# Autodesk Inventor assembly: 1.5 in Bottom Block WCP-0419
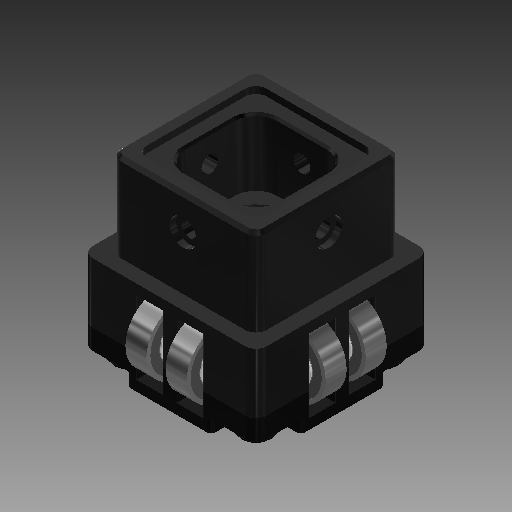
[picture p0: Inventor's stored thumbnail of the model, 512x512]
Saved by Autodesk Inventor 2023 (Build 270158000, 158)
## iProperties
Created: 2022-01-15
Part Number: 1.5 in Bottom Block WCP-0419
Document SubType Name: Assembly
Mass: 160.862 g
Surface Area: 331.6 cm^2
Volume: 41.9815 cm^3
Density: 3.83173 g/cm^3
Revision Number: ANY
## Documents named in this file (11)
- E:\Collaborative Robots\Collaborative Part Library\Elevators\GreyT Telescope\1.5 in Bottom Block WCP-0419.iam
- E:\Collaborative Robots\Collaborative Part Library\Elevators\GreyT Telescope\Mid-small Stage\WCP-0419-009 Rev1.ipt
- E:\Collaborative Robots\Collaborative Part Library\Elevators\GreyT Telescope\Mid-small Stage\WCP-0419-011 Rev1.ipt
- E:\Collaborative Robots\Collaborative Part Library\Hardware\Fasteners\Machine Screws\10-32 UNFx0.5 Button Head Cap Screw.ipt
- C:\Users\Cal\Desktop\Robotics\Design\Collaborative\Collaborative Parts Library\Hardware\Fasteners\Machine Screws.ipt
- E:\Collaborative Robots\Collaborative Part Library\Hardware\Dowel Pins\Dowel Pins\0.25in  x 0.375in Stainless Steel Dowel Pin.ipt
- C:\Users\Cal\Desktop\Robotics\Design\Collaborative\Collaborative Parts Library\Hardware\Dowel Pins\Dowel Pins.ipt
- E:\Collaborative Robots\Collaborative Part Library\Elevators\GreyT Telescope\WCP-0039 Rev1.ipt
- E:\Collaborative Robots\Collaborative Part Library\Power Transfer\Bearings and Bushings\Bearings\R4.ipt
- C:\Users\Cal\Desktop\Robotics\Design\Collaborative\Collaborative Parts Library\Power Transfer\Bearings and Bushings\Bearings.ipt
- E:\Collaborative Robots\Collaborative Part Library\Elevators\GreyT Telescope\Mid-small Stage\WCP-0419-007 Rev1.ipt
## Components (39 placed, 7 different names)
1. WCP-0419-007 Rev1:1
2. WCP-0419-009 Rev1:1 — Insert:2, Tangent:1
3. WCP-0419-011 Rev1:1 — Mate:1
4. 0.25in  x 0.375in Stainless Steel Dowel Pin:2 — Insert:10
5. WCP-0039 Rev1:20
6. R4:2 — Symmetry:3
7. WCP-0039 Rev1:19
8. 0.25in  x 0.375in Stainless Steel Dowel Pin:1 — Insert:10, Tangent:1
9. WCP-0039 Rev1:18
10. R4:1 — Symmetry:3
11. WCP-0039 Rev1:17
12. 10-32 UNFx0.5 Button Head Cap Screw:1 — Insert:2
13. 0.25in  x 0.375in Stainless Steel Dowel Pin:3
14. WCP-0039 Rev1:21
15. R4:3
16. WCP-0039 Rev1:22
17. 0.25in  x 0.375in Stainless Steel Dowel Pin:4
18. WCP-0039 Rev1:23
19. R4:4
20. WCP-0039 Rev1:24
21. 10-32 UNFx0.5 Button Head Cap Screw:2
22. 0.25in  x 0.375in Stainless Steel Dowel Pin:5
23. WCP-0039 Rev1:25
24. R4:5
25. WCP-0039 Rev1:26
26. 0.25in  x 0.375in Stainless Steel Dowel Pin:6
27. WCP-0039 Rev1:27
28. R4:6
29. WCP-0039 Rev1:28
30. 10-32 UNFx0.5 Button Head Cap Screw:3
31. 0.25in  x 0.375in Stainless Steel Dowel Pin:7
32. WCP-0039 Rev1:29
33. R4:7
34. WCP-0039 Rev1:30
35. 0.25in  x 0.375in Stainless Steel Dowel Pin:8
36. WCP-0039 Rev1:31
37. R4:8
38. WCP-0039 Rev1:32
39. 10-32 UNFx0.5 Button Head Cap Screw:4
## Component patterns: (4 elements, first: 0.25in  x 0.375in Stainless Steel Dowel Pin:2 + WCP-0039 Rev1:20 + R4:2 + WCP-0039 Rev1:19 + 0.25in  x 0.375in Stainless Steel Dowel Pin:1 + WCP-0039 Rev1:18 + R4:1 + WCP-0039 Rev1:17 + 10-32 UNFx0.5 Button Head Cap Screw:1)
## Relationships (18: Insert 7, Mate 4, Symmetry 3, Angle 2, Tangent 2)
- Mate:1: WCP-0419-011 Rev1:1
- [Mate]: WCP-0419-007 Rev1:1 ↔ WCP-0419-011 Rev1:1
- [Angle] (0 deg): WCP-0419-007 Rev1:1 ↔ WCP-0419-011 Rev1:1
- [Insert]: WCP-0419-007 Rev1:1 ↔ WCP-0419-009 Rev1:1
- [Angle] (0 deg): WCP-0419-007 Rev1:1 ↔ WCP-0419-009 Rev1:1
- Insert:2: WCP-0419-009 Rev1:1 ↔ 10-32 UNFx0.5 Button Head Cap Screw:1
- [Insert]: R4:1 ↔ WCP-0039 Rev1:17
- [Insert]: WCP-0039 Rev1:18 ↔ R4:1
- [Mate]: 0.25in  x 0.375in Stainless Steel Dowel Pin:1 ↔ R4:1
- [Symmetry]: WCP-0039 Rev1:18 ↔ WCP-0039 Rev1:17
- [Insert]: R4:2 ↔ WCP-0039 Rev1:19
- [Insert]: WCP-0039 Rev1:20 ↔ R4:2
- [Mate]: 0.25in  x 0.375in Stainless Steel Dowel Pin:2 ↔ R4:2
- [Symmetry]: WCP-0039 Rev1:20 ↔ WCP-0039 Rev1:19
- Insert:10: 0.25in  x 0.375in Stainless Steel Dowel Pin:2 ↔ 0.25in  x 0.375in Stainless Steel Dowel Pin:1
- Tangent:1: WCP-0419-009 Rev1:1 ↔ 0.25in  x 0.375in Stainless Steel Dowel Pin:1
- [Tangent]: WCP-0419-007 Rev1:1 ↔ 0.25in  x 0.375in Stainless Steel Dowel Pin:2
- Symmetry:3: R4:2 ↔ R4:1
## Named parameters: d10_d6 = 0 mm, d11_d7 = 0 mm, d12_d8 = 0 mm, d13_d6 = 0 mm, d14_d7 = 0 mm, d15_d8 = 0 mm
